# Autodesk Inventor assembly: GE-12028
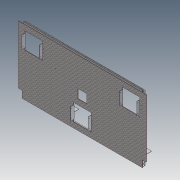
[picture p0: Inventor's stored thumbnail of the model, 180x180]
Saved by Autodesk Inventor 2012 (Build 160160000, 160)
## iProperties
Created: 2008-05-29
Part Number: GE-12028
Document SubType Name: Assembly
Designer: dfoster
Description: End Panel, Center
Title: End Panel, Center
Author: narosenberg
## Documents named in this file (7)
- C:\Data Folder\FRC 2012 Field\Components\GE-12028.iam
- C:\Data Folder\FRC 2012 Field\Components\GE-12028-01.ipt
- C:\Data Folder\FRC 2012 Field\Components\GE-12028-05.ipt
- C:\Data Folder\FRC 2012 Field\Components\GE-12028-03.ipt
- C:\Data Folder\FRC 2012 Field\Components\GE-12028-04.iam
- C:\Data Folder\FRC 2012 Field\Components\GE-12028-06.ipt
- C:\Data Folder\FRC 2012 Field\Components\GE-12028-02.ipt
## Components (14 placed, 6 different names)
1. GE-12028-01:1 — Flush:10, Mate:23, Flush:9, Flush:8, Mate:22, Flush:7, Mate:10, Flush:8, Mate:12, Mate:13, Mate:14, Mate:15, Mate:16, Mate:17, Mate:18, Mate:19, Mate:20, Mate:21, Mate:22, Mate:23, Mate:24, Mate:25, Mate:26
2. GE-12028-05:1 — Mate:11, Mate:12, Flush:10
3. GE-12028-03:1 — Flush:10, Mate:23, Flush:9, Mate:11, Flush:10
4. GE-12028-03:2 — Flush:9, Flush:8, Mate:22, Flush:11, Mate:25, Mate:24, Flush:13, Mate:29, Mate:28, Flush:9
5. GE-12028-04:1 [sub-assembly] — Flush:11, Mate:25, Mate:24, Mate:27, Mate:29, Flush:15
6. GE-12028-04:2 [sub-assembly] — Flush:13, Mate:29, Mate:28, Mate:28, Mate:30, Flush:16
7. GE-12028-06:1 — Mate:14, Mate:17, Flush:11
8. GE-12028-06:2 — Mate:13, Mate:18, Mate:21, Flush:11, Flush:12, Flush:13
9. GE-12028-06:3 — Mate:16, Mate:20, Flush:13
10. GE-12028-06:4 — Mate:15, Mate:19, Flush:12
11. GE-12028-06:5 — Mate:22, Mate:24, Flush:14
12. GE-12028-06:6 — Mate:23, Mate:25, Flush:14, Mate:26
13. GE-12028-02:1 — Mate:27, Mate:29, Flush:15
14. GE-12028-02:2 — Mate:28, Mate:30, Flush:16
## Relationships (42: Mate 27, Flush 15)
- Flush:10 (63.5 mm): GE-12028-01:1 ↔ GE-12028-03:1
- Mate:23: GE-12028-01:1 ↔ GE-12028-03:1
- Flush:9 (63.5 mm): GE-12028-01:1 ↔ GE-12028-03:2
- Flush:8: GE-12028-01:1 ↔ GE-12028-03:2
- Mate:22: GE-12028-01:1 ↔ GE-12028-03:2
- Flush:11 (-127 mm): GE-12028-03:2 ↔ GE-12028-04:1
- Mate:25: GE-12028-03:2 ↔ GE-12028-04:1
- Mate:24: GE-12028-03:2 ↔ GE-12028-04:1
- Flush:13 (127 mm): GE-12028-03:2 ↔ GE-12028-04:2
- Mate:29: GE-12028-03:2 ↔ GE-12028-04:2
- Mate:28: GE-12028-03:2 ↔ GE-12028-04:2
- Flush:7 (914.4 mm): GE-12028-01:1
- Mate:10: GE-12028-01:1
- Flush:8: GE-12028-01:1
- Flush:9 (-889 mm): GE-12028-03:1 ↔ GE-12028-03:2
- Mate:11: GE-12028-05:1 ↔ GE-12028-03:1
- Mate:12: GE-12028-01:1 ↔ GE-12028-05:1
- Flush:10: GE-12028-05:1 ↔ GE-12028-03:1
- Mate:13: GE-12028-01:1 ↔ GE-12028-06:2
- Mate:14: GE-12028-01:1 ↔ GE-12028-06:1
- Mate:15: GE-12028-01:1 ↔ GE-12028-06:4
- Mate:16: GE-12028-01:1 ↔ GE-12028-06:3
- Mate:17: GE-12028-01:1 ↔ GE-12028-06:1
- Mate:18: GE-12028-01:1 ↔ GE-12028-06:2
- Mate:19: GE-12028-01:1 ↔ GE-12028-06:4
- Mate:20: GE-12028-01:1 ↔ GE-12028-06:3
- Mate:21 (31.75 mm): GE-12028-01:1 ↔ GE-12028-06:2
- Flush:11: GE-12028-06:1 ↔ GE-12028-06:2
- Flush:12: GE-12028-06:2 ↔ GE-12028-06:4
- Flush:13: GE-12028-06:2 ↔ GE-12028-06:3
- Mate:22: GE-12028-01:1 ↔ GE-12028-06:5
- Mate:23: GE-12028-01:1 ↔ GE-12028-06:6
- Mate:24: GE-12028-01:1 ↔ GE-12028-06:5
- Mate:25: GE-12028-01:1 ↔ GE-12028-06:6
- Flush:14: GE-12028-06:5 ↔ GE-12028-06:6
- Mate:26 (31.75 mm): GE-12028-01:1 ↔ GE-12028-06:6
- Mate:27: GE-12028-04:1 ↔ GE-12028-02:1
- Mate:28: GE-12028-04:2 ↔ GE-12028-02:2
- Mate:29 (-25.4 mm): GE-12028-04:1 ↔ GE-12028-02:1
- Flush:15: GE-12028-04:1 ↔ GE-12028-02:1
- Mate:30 (-25.4 mm): GE-12028-04:2 ↔ GE-12028-02:2
- Flush:16: GE-12028-04:2 ↔ GE-12028-02:2
